# Autodesk Inventor assembly: Fixture Assembly
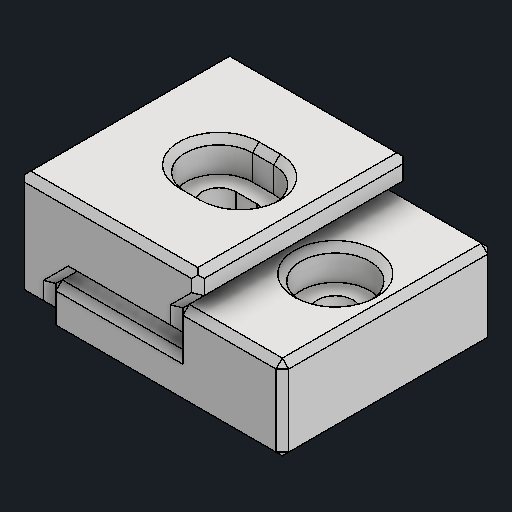
[picture p0: Inventor's stored thumbnail of the model, 512x512]
Saved by Autodesk Inventor 2026.2 (Build 302298000, 298)
## iProperties
Created: 2026-07-19
Part Number: Fixture Assembly
Document SubType Name: Assembly
Designer: JoshuaEah
Author: JoshuaEah
## Documents named in this file (3)
- C:\Users\JoshuaEah\Documents\GitHub\Designed-Trinkets\Guitar\Modular Pedalboard\Fixture Assembly.iam
- C:\Users\JoshuaEah\Documents\GitHub\Designed-Trinkets\Guitar\Modular Pedalboard\Part1.ipt
- C:\Users\JoshuaEah\Documents\GitHub\Designed-Trinkets\Guitar\Modular Pedalboard\Part2.ipt
## Components (2 placed, 2 different names)
1. Part1:1 — Flush:1, Transitional:1, Transitional:2
2. Part2:1 — Flush:1, Transitional:1, Transitional:2
## Relationships (3: Transitional 2, Flush 1)
- Flush:1: Part1:1 ↔ Part2:1
- Transitional:1: Part1:1 ↔ Part2:1
- Transitional:2: Part1:1 ↔ Part2:1
